# Autodesk Inventor assembly: MiddleBackTube
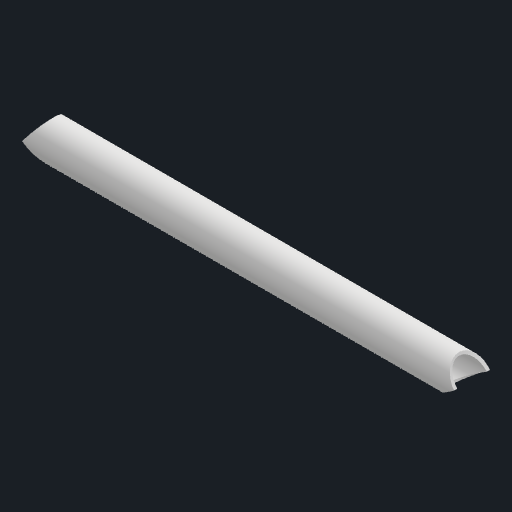
[picture p0: Inventor's stored thumbnail of the model, 512x512]
Saved by Autodesk Inventor 2025.2 (Build 292293000, 293)
## iProperties
Created: 2025-04-01
Part Number: MiddleBackTube
Document SubType Name: Assembly
Designer: valer
Author: valer
## Documents named in this file (2)
- C:\Users\valer\Desktop\str1ker\cad\MiddleBackTube.iam
- C:\Users\valer\Desktop\str1ker\cad\ChestMiddleBackTube.ipt
## Components (1 placed, 1 different names)
1. ChestMiddleBackTube:1 — Mate:1
## Relationships (1: Mate 1)
- Mate:1: ChestMiddleBackTube:1
